# Autodesk Inventor assembly: HS 36T Gear, No Insert
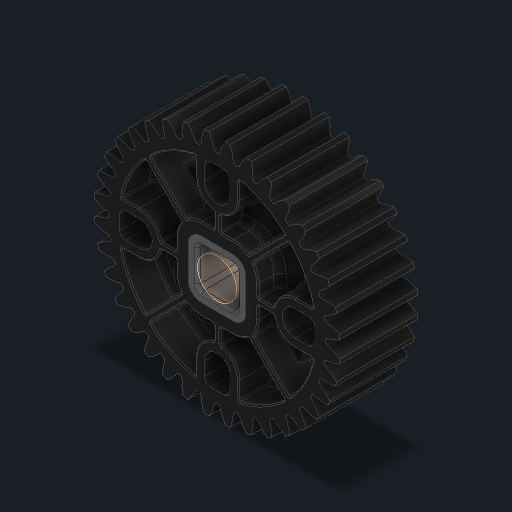
[picture p0: Inventor's stored thumbnail of the model, 512x512]
Saved by Autodesk Inventor 2025.1 (Build 291241000, 241)
## iProperties
Created: 2022-08-02
Part Number: HS 36T Gear, No Insert
Document SubType Name: Assembly
Designer: avere
Author: ylu12
## Documents named in this file (2)
- C:\Users\avere\VEX\High Stakes\CAD\V4\Chassis\Drivebay Right\HS 36T Gear, No Insert.iam
- C:\Users\avere\VEX\High Stakes\CAD\V4\Chassis\Drivebay Right\HS 36T Gear, No Insert.ipt
## Components (1 placed, 1 different names)
1. HS 36T Gear, No Insert:1 — Mate:10, Mate:9, Flush:5
## Relationships (3: Mate 2, Flush 1)
- Mate:10: HS 36T Gear, No Insert:1
- Mate:9: HS 36T Gear, No Insert:1
- Flush:5: HS 36T Gear, No Insert:1
